# Autodesk Inventor assembly: ensamble_griper
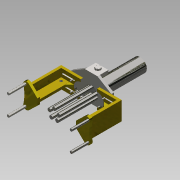
[picture p0: Inventor's stored thumbnail of the model, 180x180]
Saved by Autodesk Inventor 2021 (Build 250183000, 183)
## iProperties
Created: 2022-01-31
Part Number: ensamble_griper
Document SubType Name: Assembly
Designer: Osmar Ediber Toloza Bernal
Mass: 244358 g
Surface Area: 19842 cm^2
Volume: 30544.8 cm^3
Density: 8 g/cm^3
Author: Osmar Ediber Toloza Bernal
## Documents named in this file (5)
- H:\Mi unidad\2021 2\Robotica\Proyecto\modelado\griper\ensamble_griper.iam
- H:\Mi unidad\2021 2\Robotica\Proyecto\modelado\griper\soporte.ipt
- H:\Mi unidad\2021 2\Robotica\Proyecto\modelado\griper\garra_griper.ipt
- H:\Mi unidad\2021 2\Robotica\Proyecto\modelado\griper\garra_griper_MIR.ipt
- H:\Mi unidad\2021 2\Robotica\Proyecto\modelado\griper\atornillador.ipt
## Components (4 placed, 4 different names)
1. soporte:1 — Coincidencia:1, Coincidencia:2, Coincidencia:7, Tangente:1, Coincidencia:4, Tangente:2, Coincidencia:5, Tangente:3, Tangente:4, Coincidencia:6, Rígido:1
2. garra_griper:1 — Tangente:1, Coincidencia:5, Tangente:3, Coincidencia:6
3. garra_griper_MIR:1 — Coincidencia:4, Tangente:2, Tangente:4
4. atornillador:1 — Rígido:1
## Relationships (11: Mate 6, Tangent 4, WeldJoint 1)
- Coincidencia:1 [Mate]: soporte:1
- Coincidencia:2 [Mate]: soporte:1
- Coincidencia:7 [Mate] (50 mm): soporte:1
- Tangente:1: soporte:1 ↔ garra_griper:1
- Coincidencia:4 [Mate]: soporte:1 ↔ garra_griper_MIR:1
- Tangente:2: soporte:1 ↔ garra_griper_MIR:1
- Coincidencia:5 [Mate]: soporte:1 ↔ garra_griper:1
- Tangente:3: soporte:1 ↔ garra_griper:1
- Tangente:4: soporte:1 ↔ garra_griper_MIR:1
- Coincidencia:6 [Mate]: soporte:1 ↔ garra_griper:1
- Rígido:1 [WeldJoint]: soporte:1 ↔ atornillador:1
